# Autodesk Inventor assembly: SHOOTING Assembly
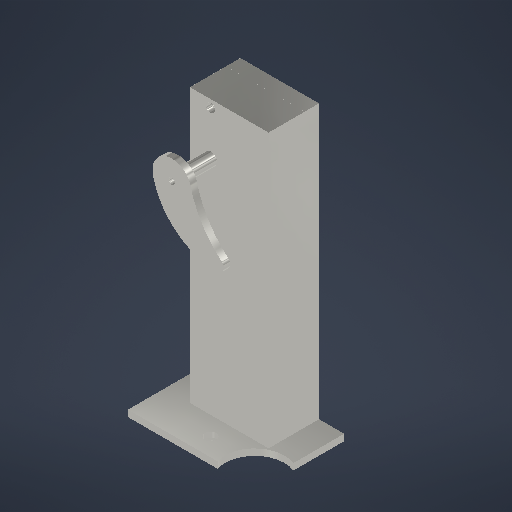
[picture p0: Inventor's stored thumbnail of the model, 512x512]
Saved by Autodesk Inventor 2026.2 (Build 302298010, 298A)
## iProperties
Created: 2026-04-19
Part Number: SHOOTING Assembly
Document SubType Name: Assembly
Designer: lenovo
Author: lenovo
## Documents named in this file (7)
- F:\Semester 4\Basics of Mechatronics\Final\SHOOTING Assembly.0002.iam
- F:\Semester 4\Basics of Mechatronics\Final\Housing of DC Motor.ipt
- F:\Semester 4\Basics of Mechatronics\Final\Cover of DC Housing.ipt
- F:\Semester 4\Basics of Mechatronics\Final\DC - Gear Box Motor.ipt
- F:\Semester 4\Basics of Mechatronics\Final\encoder disk.ipt
- F:\Semester 4\Basics of Mechatronics\Final\Interrupt Sensor.ipt
- F:\Semester 4\Basics of Mechatronics\Final\p2.ipt
## Components (6 placed, 6 different names)
1. Housing of DC Motor:1 — Mate:2, Mate:5, Mate:6, Mate:7, Mate:8
2. DC - Gear Box Motor:3 — Mate:2, Mate:3, Tangent:1
3. encoder disk:1 — Mate:3, Mate:4
4. Interrupt Sensor:1 — Mate:4
5. Cover of DC Housing:1 — Tangent:1, Mate:5, Mate:6
6. Shooter:1 — Mate:7, Mate:8
## Relationships (8: Mate 7, Tangent 1)
- Mate:2: Housing of DC Motor:1 ↔ DC - Gear Box Motor:3
- Mate:3: DC - Gear Box Motor:3 ↔ encoder disk:1
- Mate:4: encoder disk:1 ↔ Interrupt Sensor:1
- Tangent:1: DC - Gear Box Motor:3 ↔ Cover of DC Housing:1
- Mate:5: Housing of DC Motor:1 ↔ Cover of DC Housing:1
- Mate:6: Housing of DC Motor:1 ↔ Cover of DC Housing:1
- Mate:7: Housing of DC Motor:1 ↔ Shooter:1
- Mate:8: Housing of DC Motor:1 ↔ Shooter:1
## Named parameters: Finish1_Area = 1258.99, Finish1_Thickness = 0.05 mm
note: some values were not read from the file. Shown as the stored number, unit unknown: "Finish1_Area".
